# Autodesk Inventor assembly: Rb PEEK
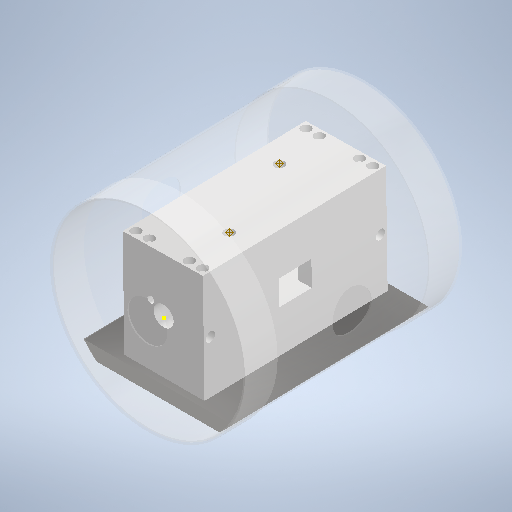
[picture p0: Inventor's stored thumbnail of the model, 512x512]
Saved by Autodesk Inventor 2025.1 (Build 291241000, 241)
## iProperties
Created: 2025-05-09
Part Number: Rb PEEK
Document SubType Name: Assembly
Designer: E. Moreno
Author: E. Moreno
Title: Rb PEEK - Ensamblado
## Documents named in this file (19)
- C:\Users\dell 5810\Documents\M\GitHub\LAFriOC\Rb oven\Rb PEEK\Rb Full Modificación.iam
- C:\Users\dell 5810\Documents\M\GitHub\LAFriOC\Rb oven\Rb PEEK\Rb PEEK - Arriba.ipt
- C:\Users\dell 5810\Documents\M\GitHub\LAFriOC\Rb oven\Rb PEEK\Rb PEEK - Largo.ipt
- C:\Users\dell 5810\Documents\M\GitHub\LAFriOC\Rb oven\Rb PEEK\Rb PEEK - Corto con ventana.ipt
- C:\Users\dell 5810\Documents\M\GitHub\LAFriOC\Rb oven\Rb PEEK\Rb PEEK - Soporte.ipt
- C:\Users\dell 5810\Documents\M\GitHub\LAFriOC\Rb oven\Rb PEEK\Rb PEEK - Abajo.ipt
- E:\Users\USER\Documents\Inventor\Content Center Files\R2025\en-US\AS 1420\AS 1420 - 1973 - M4 x 8.ipt
- C:\Users\dell 5810\Documents\M\GitHub\LAFriOC\Rb oven\Rb parts\Cell.ipt
- E:\Users\USER\Documents\Inventor\Content Center Files\R2025\en-US\AS 1420\AS 1420 - 1973 - M4 x 25.ipt
- E:\Users\USER\Documents\Inventor\Content Center Files\R2025\en-US\AS 1420\AS 1420 - 1973 - M4 x 12.ipt
- C:\Users\dell 5810\Documents\M\GitHub\LAFriOC\Rb oven\MS-1L Shield\Shield.iam
- E:\Users\USER\Documents\Inventor\Content Center Files\R2025\en-US\AS 1420\AS 1420 - 1973 - M6 x 16.ipt
- C:\Users\dell 5810\Documents\M\GitHub\LAFriOC\Rb oven\Rb PEEK\Rb PEEK - Largo_MIR.ipt
- C:\Users\dell 5810\Documents\M\GitHub\LAFriOC\Rb oven\Rb parts\Thermistor.ipt
- C:\Users\dell 5810\Documents\M\GitHub\LAFriOC\Rb oven\Rb oven housing\Modificación\Rb oven housing - Bottom.iam
- C:\Users\dell 5810\Documents\M\GitHub\LAFriOC\Rb oven\Rb oven housing\Modificación\Rb oven housing - Top.iam
- C:\Users\dell 5810\Documents\M\GitHub\LAFriOC\Rb oven\Rb parts\Heater4.ipt
- C:\Users\dell 5810\Documents\M\GitHub\LAFriOC\Rb oven\Rb PEEK\Rb Full Modificación\AIP\Cable y arnés\Heater4 Cable1.iam
- C:\Users\dell 5810\Documents\M\GitHub\LAFriOC\Rb oven\Rb PEEK\Rb Full Modificación\AIP\Cable y arnés\Heater4 Cable2.iam
## Components (48 placed, 18 different names)
1. Shield:1 [sub-assembly] — Coincidencia:41
2. Heater4:1 — Insertar:36
3. Heater4:2 — Insertar:37
4. Heater4 Cable1 [sub-assembly]
5. Heater4 Cable2 [sub-assembly]
6. AS 1420 - Metric M6 x 16:1 — Insert:33
7. AS 1420 - Metric M6 x 16:2 — Insert:34
8. Thermistor:1
9. Thermistor:2
10. Rb PEEK - Arriba:1 — Coincidencia:1, Coincidencia:2, Coincidencia:3, Coincidencia:5, Coincidencia:6, Coincidencia:33, Insert:9, Insert:10, Insert:11, Insert:12, Insert:13, Insert:14, Insert:15, Insert:16
11. Rb PEEK - Abajo:1 — Coincidencia:21, Coincidencia:22, Coincidencia:23, Coincidencia:29, Coincidencia:30, Coincidencia:34, Insert:21, Insert:24, Insert:25, Insert:26, Insert:27, Insert:28, Insert:29, Insert:30, Insert:31, Insert:32, Insert:33, Insert:34, Coincidencia:38, Coincidencia:39, Coincidencia:41
12. Rb PEEK - Largo:1 — Coincidencia:1, Coincidencia:2, Coincidencia:3, Coincidencia:4, Coincidencia:18, Coincidencia:20, Coincidencia:21, Coincidencia:22, Coincidencia:23, Insert:17, Insert:18
13. Rb PEEK - Largo_MIR:1 — Coincidencia:38, Coincidencia:39
14. Rb PEEK - Corto con ventana:1 — Coincidencia:4, Coincidencia:5, Coincidencia:6
15. Rb PEEK - Corto con ventana:2 — Coincidencia:18, Coincidencia:20, Coincidencia:33, Coincidencia:34
16. Rb PEEK - Soporte:1 — Coincidencia:29, Insert:1, Coincidencia:40
17. Rb PEEK - Soporte:2 — Coincidencia:30, Insert:2
18. Rb oven housing - Top:1 [sub-assembly] — Insertar:35
19. Rb oven housing - Bottom:1 [sub-assembly] — Coincidencia:40, Insertar:36, Insertar:37
20. Cell:1 — Insertar:35
21. AS 1420 - Metric M4 x 8:1 — Insert:1
22. AS 1420 - Metric M4 x 8:2 — Insert:2
23. AS 1420 - Metric M4 x 25:1
24. AS 1420 - Metric M4 x 25:2
25. AS 1420 - Metric M4 x 25:3
26. AS 1420 - Metric M4 x 25:4
27. AS 1420 - Metric M4 x 25:5 — Insert:9
28. AS 1420 - Metric M4 x 25:6 — Insert:10
29. AS 1420 - Metric M4 x 25:7 — Insert:11
30. AS 1420 - Metric M4 x 25:8 — Insert:12
31. AS 1420 - Metric M4 x 25:9 — Insert:13
32. AS 1420 - Metric M4 x 25:10 — Insert:14
33. AS 1420 - Metric M4 x 25:11 — Insert:15
34. AS 1420 - Metric M4 x 25:12 — Insert:16
35. AS 1420 - Metric M4 x 12:3 — Insert:17
36. AS 1420 - Metric M4 x 12:4 — Insert:18
37. AS 1420 - Metric M4 x 12:5
38. AS 1420 - Metric M4 x 12:6
39. AS 1420 - Metric M4 x 25:13 — Insert:21
40. AS 1420 - Metric M4 x 25:14 — Insert:24
41. AS 1420 - Metric M4 x 25:15 — Insert:25
42. AS 1420 - Metric M4 x 25:16 — Insert:26
43. AS 1420 - Metric M4 x 25:17 — Insert:27
44. AS 1420 - Metric M4 x 25:18 — Insert:28
45. AS 1420 - Metric M4 x 25:19 — Insert:29
46. AS 1420 - Metric M4 x 25:20 — Insert:30
47. AS 1420 - Metric M4 x 12:1 — Insert:31
48. AS 1420 - Metric M4 x 12:2 — Insert:32
## Relationships (46: Insert 27, Mate 19)
- Coincidencia:1 [Mate]: Rb PEEK - Arriba:1 ↔ Rb PEEK - Largo:1
- Coincidencia:2 [Mate]: Rb PEEK - Arriba:1 ↔ Rb PEEK - Largo:1
- Coincidencia:3 [Mate]: Rb PEEK - Arriba:1 ↔ Rb PEEK - Largo:1
- Coincidencia:4 [Mate]: Rb PEEK - Largo:1 ↔ Rb PEEK - Corto con ventana:1
- Coincidencia:5 [Mate]: Rb PEEK - Arriba:1 ↔ Rb PEEK - Corto con ventana:1
- Coincidencia:6 [Mate]: Rb PEEK - Arriba:1 ↔ Rb PEEK - Corto con ventana:1
- Coincidencia:18 [Mate]: Rb PEEK - Largo:1 ↔ Rb PEEK - Corto con ventana:2
- Coincidencia:20 [Mate]: Rb PEEK - Largo:1 ↔ Rb PEEK - Corto con ventana:2
- Coincidencia:21 [Mate]: Rb PEEK - Abajo:1 ↔ Rb PEEK - Largo:1
- Coincidencia:22 [Mate]: Rb PEEK - Abajo:1 ↔ Rb PEEK - Largo:1
- Coincidencia:23 [Mate]: Rb PEEK - Abajo:1 ↔ Rb PEEK - Largo:1
- Coincidencia:29 [Mate]: Rb PEEK - Abajo:1 ↔ Rb PEEK - Soporte:1
- Coincidencia:30 [Mate]: Rb PEEK - Abajo:1 ↔ Rb PEEK - Soporte:2
- Insert:1: Rb PEEK - Soporte:1 ↔ AS 1420 - Metric M4 x 8:1
- Insert:2: Rb PEEK - Soporte:2 ↔ AS 1420 - Metric M4 x 8:2
- Coincidencia:33 [Mate]: Rb PEEK - Arriba:1 ↔ Rb PEEK - Corto con ventana:2
- Coincidencia:34 [Mate]: Rb PEEK - Abajo:1 ↔ Rb PEEK - Corto con ventana:2
- Insert:9: Rb PEEK - Arriba:1 ↔ AS 1420 - Metric M4 x 25:5
- Insert:10: Rb PEEK - Arriba:1 ↔ AS 1420 - Metric M4 x 25:6
- Insert:11: Rb PEEK - Arriba:1 ↔ AS 1420 - Metric M4 x 25:7
- Insert:12: Rb PEEK - Arriba:1 ↔ AS 1420 - Metric M4 x 25:8
- Insert:13: Rb PEEK - Arriba:1 ↔ AS 1420 - Metric M4 x 25:9
- Insert:14: Rb PEEK - Arriba:1 ↔ AS 1420 - Metric M4 x 25:10
- Insert:15: Rb PEEK - Arriba:1 ↔ AS 1420 - Metric M4 x 25:11
- Insert:16: Rb PEEK - Arriba:1 ↔ AS 1420 - Metric M4 x 25:12
- Insert:17: Rb PEEK - Largo:1 ↔ AS 1420 - Metric M4 x 12:3
- Insert:18: Rb PEEK - Largo:1 ↔ AS 1420 - Metric M4 x 12:4
- Insert:21: Rb PEEK - Abajo:1 ↔ AS 1420 - Metric M4 x 25:13
- Insert:24: Rb PEEK - Abajo:1 ↔ AS 1420 - Metric M4 x 25:14
- Insert:25: Rb PEEK - Abajo:1 ↔ AS 1420 - Metric M4 x 25:15
- Insert:26: Rb PEEK - Abajo:1 ↔ AS 1420 - Metric M4 x 25:16
- Insert:27: Rb PEEK - Abajo:1 ↔ AS 1420 - Metric M4 x 25:17
- Insert:28: Rb PEEK - Abajo:1 ↔ AS 1420 - Metric M4 x 25:18
- Insert:29: Rb PEEK - Abajo:1 ↔ AS 1420 - Metric M4 x 25:19
- Insert:30: Rb PEEK - Abajo:1 ↔ AS 1420 - Metric M4 x 25:20
- Insert:31: Rb PEEK - Abajo:1 ↔ AS 1420 - Metric M4 x 12:1
- Insert:32: Rb PEEK - Abajo:1 ↔ AS 1420 - Metric M4 x 12:2
- Insert:33: AS 1420 - Metric M6 x 16:1 ↔ Rb PEEK - Abajo:1
- Insert:34: AS 1420 - Metric M6 x 16:2 ↔ Rb PEEK - Abajo:1
- Coincidencia:38 [Mate]: Rb PEEK - Abajo:1 ↔ Rb PEEK - Largo_MIR:1
- Coincidencia:39 [Mate]: Rb PEEK - Abajo:1 ↔ Rb PEEK - Largo_MIR:1
- Coincidencia:40 [Mate]: Rb PEEK - Soporte:1 ↔ Rb oven housing - Bottom:1
- Insertar:35 (-80 mm): Rb oven housing - Top:1 ↔ Cell:1
- Insertar:36 (-10.5 mm): Heater4:1 ↔ Rb oven housing - Bottom:1
- Insertar:37 (-10.5 mm): Heater4:2 ↔ Rb oven housing - Bottom:1
- Coincidencia:41 [Mate]: Shield:1 ↔ Rb PEEK - Abajo:1
